# Autodesk Inventor assembly: theMonarchBoxAssembly
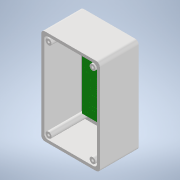
[picture p0: Inventor's stored thumbnail of the model, 180x180]
Saved by Autodesk Inventor 2020 (Build 240168000, 168)
## iProperties
Created: 2020-10-14
Part Number: theMonarchBoxAssembly
Document SubType Name: Assembly
Designer: s4393944
Author: s4393944
## Documents named in this file (3)
- \\puffball.labs.eait.uq.edu.au\s4393944\Desktop\THESIS\PCB\PCBHolders\theMonarchBoxAssembly.iam
- \\puffball.labs.eait.uq.edu.au\s4393944\Desktop\THESIS\PCB\PCBHolders\theMonarchPCBHolder.ipt
- \\puffball.labs.eait.uq.edu.au\s4393944\Desktop\THESIS\PCB\theMonarchTransmitter\theMonarchTransmitter.iam
## Components (2 placed, 2 different names)
1. theMonarchPCBHolder:1 — Mate:1, Mate:2, Mate:3
2. theMonarchTransmitter:1 [sub-assembly] — Mate:1, Mate:2, Mate:3
## Relationships (3: Mate 3)
- Mate:1: theMonarchPCBHolder:1 ↔ theMonarchTransmitter:1
- Mate:2: theMonarchPCBHolder:1 ↔ theMonarchTransmitter:1
- Mate:3: theMonarchPCBHolder:1 ↔ theMonarchTransmitter:1
